# Autodesk Inventor assembly: Carriage_Assembly
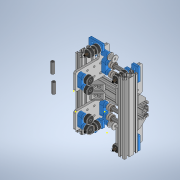
[picture p0: Inventor's stored thumbnail of the model, 180x180]
Saved by Autodesk Inventor 2021 (Build 250183000, 183)
## iProperties
Created: 2021-09-08
Part Number: Carriage_Assembly
Document SubType Name: Assembly
Designer: Jorian Brusind
Author: Jorian Brusind
## Documents named in this file (10)
- C:\Users\Jorian Brusind\Documents\GitHub\PersonalProjects\HyperRail\Inventor Files\Carriage_Assembly.iam
- C:\Users\Jorian Brusind\Documents\GitHub\PersonalProjects\Inventor Projects\Useful models\8020_Sets\IPT_20_Series\IPT_20_Series\20-2040_200mm.ipt
- C:\Users\Jorian Brusind\Documents\GitHub\PersonalProjects\Inventor Projects\Useful models\8020_Sets\IPT_20_Series\IPT_20_Series\20-2040_150mm.ipt
- C:\Users\Jorian Brusind\Documents\GitHub\PersonalProjects\HyperRail\Inventor Files\X_CarriageL_V2_0_Short.iam
- C:\Users\Jorian Brusind\Documents\GitHub\PersonalProjects\HyperRail\Inventor Files\X_CarriageR_V2_0_Short.iam
- C:\Users\Jorian Brusind\Documents\GitHub\PersonalProjects\HyperRail\Inventor Files\X_CarriageR_V2_0.iam
- C:\Users\Jorian Brusind\Documents\GitHub\PersonalProjects\HyperRail\Inventor Files\X_Carriage_V2_0.iam
- C:\Users\Jorian Brusind\Documents\GitHub\PersonalProjects\Inventor Projects\Useful models\8020_Sets\IPT_20_Series\Extra_20_Series\8020_14056m\14056_m.ipt
- C:\Users\Jorian Brusind\Documents\GitHub\PersonalProjects\HyperRail\Inventor Files\Buffer.iam
- C:\Users\Jorian Brusind\Documents\GitHub\PersonalProjects\Inventor Projects\Useful models\Metric Spacer_Standoffs\hex spacer standoff nut M5 L30.ipt
## Components (23 placed, 9 different names)
1. 20-2040_200mm:1 — Mate:1, Flush:1, Mate:2, Flush:2, Mate:3, Mate:4, Mate:5, Mate:6, Mate:7, Flush:3, Mate:9, Flush:6, Flush:7, Flush:11, Flush:12, Mate:24, Mate:25, Mate:29, Mate:51, Flush:18, Mate:53, Flush:22
2. 20-2040_200mm:2 — Mate:10, Mate:11, Flush:5, Mate:12, Mate:13, Flush:6, Flush:7, Mate:18, Mate:19, Flush:9, Flush:10, Mate:52, Flush:20, Flush:21, Mate:56, Flush:23
3. 20-2040_150mm:1 — Flush:3, Mate:8, Mate:9, Mate:20, Mate:21, Mate:22, Mate:23, Mate:26, Flush:14, Mate:27, Flush:15
4. X_CarriageL_V2_0_Short:1 [sub-assembly] — Mate:10, Flush:5, Mate:13, Mate:57, Mate:65, Mate:68
5. X_CarriageR_V2_0_Short:1 [sub-assembly] — Mate:11, Mate:12, Mate:59, Mate:60, Mate:63
6. X_CarriageR_V2_0:1 [sub-assembly] — Mate:1, Flush:1, Mate:2, Mate:8, Mate:54, Mate:64, Mate:66, Mate:67
7. X_Carriage_V2_0:1 [sub-assembly] — Flush:2, Mate:3, Mate:4, Mate:55, Mate:58, Mate:61, Mate:62
8. 14056_m:1 — Mate:19, Mate:21, Flush:9
9. 14056_m:2 — Mate:18, Mate:20, Flush:10
10. 14056_m:3 — Mate:22, Flush:12, Flush:13
11. 14056_m:4 — Mate:23, Flush:11, Flush:13, Mate:24
12. 14056_m:5 — Mate:27, Mate:29, Flush:15
13. 14056_m:6 — Mate:25, Mate:26, Flush:14
14. Buffer:1 [sub-assembly] — Mate:56, Flush:23, Mate:57
15. Buffer:2 [sub-assembly] — Mate:53, Flush:22, Mate:54
16. Buffer:3 [sub-assembly] — Mate:52, Flush:20, Flush:21
17. Buffer:4 [sub-assembly] — Mate:51, Flush:18, Mate:55
18. hex spacer standoff nut M5 L30:1
19. hex spacer standoff nut M5 L30:2 — Mate:64, Mate:65, Mate:66
20. hex spacer standoff nut M5 L30:3 — Mate:67, Mate:68
21. hex spacer standoff nut M5 L30:4 — Mate:62, Mate:63
22. hex spacer standoff nut M5 L30:5
23. hex spacer standoff nut M5 L30:6 — Mate:58, Mate:59, Mate:60, Mate:61
## Relationships (60: Mate 42, Flush 18)
- Mate:1: 20-2040_200mm:1 ↔ X_CarriageR_V2_0:1
- Flush:1: 20-2040_200mm:1 ↔ X_CarriageR_V2_0:1
- Mate:2 (5 mm): 20-2040_200mm:1 ↔ X_CarriageR_V2_0:1
- Flush:2: 20-2040_200mm:1 ↔ X_Carriage_V2_0:1
- Mate:3: 20-2040_200mm:1 ↔ X_Carriage_V2_0:1
- Mate:4 (5 mm): 20-2040_200mm:1 ↔ X_Carriage_V2_0:1
- Mate:5: 20-2040_200mm:1
- Mate:6: 20-2040_200mm:1
- Mate:7: 20-2040_200mm:1
- Flush:3: 20-2040_200mm:1 ↔ 20-2040_150mm:1
- Mate:8 (5 mm): 20-2040_150mm:1 ↔ X_CarriageR_V2_0:1
- Mate:9 (5 mm): 20-2040_200mm:1 ↔ 20-2040_150mm:1
- Mate:10: 20-2040_200mm:2 ↔ X_CarriageL_V2_0_Short:1
- Mate:11: 20-2040_200mm:2 ↔ X_CarriageR_V2_0_Short:1
- Flush:5: 20-2040_200mm:2 ↔ X_CarriageL_V2_0_Short:1
- Mate:12 (3 mm): 20-2040_200mm:2 ↔ X_CarriageR_V2_0_Short:1
- Mate:13 (3 mm): 20-2040_200mm:2 ↔ X_CarriageL_V2_0_Short:1
- Flush:6: 20-2040_200mm:1 ↔ 20-2040_200mm:2
- Flush:7: 20-2040_200mm:1 ↔ 20-2040_200mm:2
- Mate:18: 20-2040_200mm:2 ↔ 14056_m:2
- Mate:19: 20-2040_200mm:2 ↔ 14056_m:1
- Mate:20: 20-2040_150mm:1 ↔ 14056_m:2
- Mate:21: 20-2040_150mm:1 ↔ 14056_m:1
- Flush:9: 20-2040_200mm:2 ↔ 14056_m:1
- Flush:10: 20-2040_200mm:2 ↔ 14056_m:2
- Mate:22: 20-2040_150mm:1 ↔ 14056_m:3
- Mate:23: 20-2040_150mm:1 ↔ 14056_m:4
- Flush:11: 20-2040_200mm:1 ↔ 14056_m:4
- Flush:12: 20-2040_200mm:1 ↔ 14056_m:3
- Flush:13: 14056_m:3 ↔ 14056_m:4
- Mate:24: 20-2040_200mm:1 ↔ 14056_m:4
- Mate:25: 20-2040_200mm:1 ↔ 14056_m:6
- Mate:26: 20-2040_150mm:1 ↔ 14056_m:6
- Flush:14: 20-2040_150mm:1 ↔ 14056_m:6
- Mate:27: 20-2040_150mm:1 ↔ 14056_m:5
- Mate:29: 20-2040_200mm:1 ↔ 14056_m:5
- Flush:15: 20-2040_150mm:1 ↔ 14056_m:5
- Mate:51: 20-2040_200mm:1 ↔ Buffer:4
- Flush:18: 20-2040_200mm:1 ↔ Buffer:4
- Mate:52: 20-2040_200mm:2 ↔ Buffer:3
- Flush:20: 20-2040_200mm:2 ↔ Buffer:3
- Flush:21: 20-2040_200mm:2 ↔ Buffer:3
- Mate:53: 20-2040_200mm:1 ↔ Buffer:2
- Flush:22: 20-2040_200mm:1 ↔ Buffer:2
- Mate:54: X_CarriageR_V2_0:1 ↔ Buffer:2
- Mate:55: X_Carriage_V2_0:1 ↔ Buffer:4
- Mate:56: 20-2040_200mm:2 ↔ Buffer:1
- Flush:23: 20-2040_200mm:2 ↔ Buffer:1
- Mate:57: X_CarriageL_V2_0_Short:1 ↔ Buffer:1
- Mate:58: X_Carriage_V2_0:1 ↔ hex spacer standoff nut M5 L30:6
- Mate:59: X_CarriageR_V2_0_Short:1 ↔ hex spacer standoff nut M5 L30:6
- Mate:60: X_CarriageR_V2_0_Short:1 ↔ hex spacer standoff nut M5 L30:6
- Mate:61: X_Carriage_V2_0:1 ↔ hex spacer standoff nut M5 L30:6
- Mate:62: X_Carriage_V2_0:1 ↔ hex spacer standoff nut M5 L30:4
- Mate:63: X_CarriageR_V2_0_Short:1 ↔ hex spacer standoff nut M5 L30:4
- Mate:64: X_CarriageR_V2_0:1 ↔ hex spacer standoff nut M5 L30:2
- Mate:65: X_CarriageL_V2_0_Short:1 ↔ hex spacer standoff nut M5 L30:2
- Mate:66: X_CarriageR_V2_0:1 ↔ hex spacer standoff nut M5 L30:2
- Mate:67: X_CarriageR_V2_0:1 ↔ hex spacer standoff nut M5 L30:3
- Mate:68: X_CarriageL_V2_0_Short:1 ↔ hex spacer standoff nut M5 L30:3
